# Autodesk Inventor assembly: ude
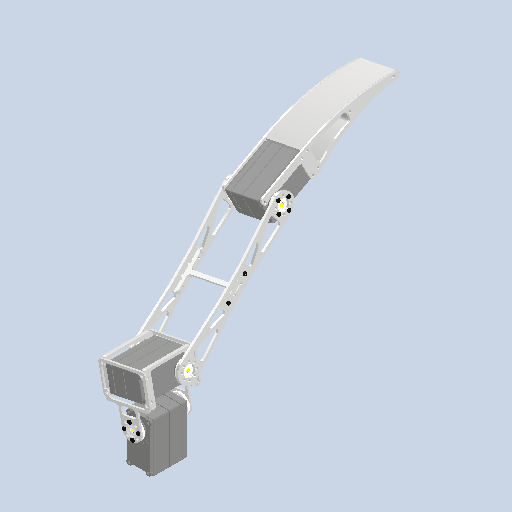
[picture p0: Inventor's stored thumbnail of the model, 512x512]
Saved by Autodesk Inventor 2024 (Build 280153000, 153)
## iProperties
Created: 2023-03-29
Part Number: ude
Document SubType Name: Assembly
Designer: right
Mass: 174.923 g
Surface Area: 565.861 cm^2
Volume: 110.018 cm^3
Density: 1.58994 g/cm^3
Author: right
## Documents named in this file (11)
- C:\Users\right\OneDrive\ドキュメント\Inventor\V2二足Light＿仮\ude.iam
- C:\Users\right\OneDrive\ドキュメント\Inventor\V2二足Light＿仮\KRS2500_scale.ipt
- C:\Users\right\OneDrive\ドキュメント\Inventor\V2二足Light＿仮\02157_SmallDiameterHornB.ipt
- C:\Users\right\OneDrive\ドキュメント\Inventor\V2二足Light＿仮\kata.ipt
- C:\Users\right\OneDrive\ドキュメント\Inventor\V2二足Light＿仮\腕.ipt
- C:\Users\right\OneDrive\ドキュメント\Inventor\V2二足Light＿仮\腕の筋交い.ipt
- C:\Users\right\OneDrive\ドキュメント\Inventor\V2二足Light＿仮\02159_SmallFreeHornC.ipt
- C:\Users\right\OneDrive\ドキュメント\Inventor\V2二足Light＿仮\hand.ipt
- C:\Users\right\OneDrive\ドキュメント\Inventor\V2二足Light＿仮\M2小ねじ.ipt
- C:\Users\right\OneDrive\ドキュメント\Inventor\V2二足Light＿仮\上腕.ipt
- C:\Users\right\OneDrive\ドキュメント\Inventor\V2二足Light＿仮\sphand2.ipt
## Components (35 placed, 10 different names)
1. KRS2500_scale:1 — 挿入:1, 挿入:63
2. 02157_SmallDiameterHornB:1 — 挿入:1, 挿入:4, 挿入:5
3. kata:1 — 挿入:4, 挿入:5, 挿入:53, 挿入:54, 挿入:55, 挿入:56, 挿入:66, 挿入:67, 挿入:71
4. KRS2500_scale:2 — 挿入:17, 挿入:69, 挿入:70, 挿入:73, 挿入:74
5. 02157_SmallDiameterHornB:2 — 挿入:15, 挿入:16
6. 腕:1 — 挿入:18, 挿入:19, 挿入:20, 挿入:21, 挿入:27, 挿入:28, 挿入:43, 挿入:44, 挿入:49, 挿入:50, 挿入:51, 挿入:52
7. 腕:2 — 挿入:15, 挿入:16, 挿入:22, 挿入:25, 挿入:26, 挿入:37, 挿入:38, 挿入:39, 挿入:40, 挿入:41, 挿入:42
8. 腕の筋交い:1 — 挿入:20, 挿入:21, 挿入:22
9. 02159_SmallFreeHornC:1 — 挿入:17, 挿入:18, 挿入:19
10. KRS2500_scale:3 — 挿入:29, 挿入:30, 挿入:31, 挿入:32
11. 02157_SmallDiameterHornB:3 — 挿入:25, 挿入:26
12. 02159_SmallFreeHornC:2 — 挿入:27, 挿入:28
13. hand:1 — 挿入:29, 挿入:30, フラッシュ:1, 挿入:75
14. hand:2 — 挿入:31, 挿入:32, 挿入:76
15. M2小ねじ:2 — 挿入:52
16. M2小ねじ:3 — 挿入:37
17. M2小ねじ:4 — 挿入:38
18. M2小ねじ:7 — 挿入:49
19. M2小ねじ:8 — 挿入:50
20. M2小ねじ:10 — 挿入:44
21. M2小ねじ:12 — 挿入:51
22. M2小ねじ:13 — 挿入:40
23. M2小ねじ:14 — 挿入:41
24. M2小ねじ:18 — 挿入:42
25. M2小ねじ:19 — 挿入:43
26. M2小ねじ:20 — 挿入:39
27. M2小ねじ:21 — 挿入:56
28. M2小ねじ:22 — 挿入:55
29. M2小ねじ:23 — 挿入:54
30. M2小ねじ:24 — 挿入:53
31. 02159_SmallFreeHornC:3 — 挿入:63, 挿入:64, 挿入:65
32. kata:2 — 挿入:64, 挿入:65, 挿入:68, 挿入:72
33. 上腕:1 — 挿入:66, 挿入:67, 挿入:68, 挿入:69, 挿入:70
34. 上腕:2 — 挿入:71, 挿入:72, 挿入:73, 挿入:74
35. sphand2:1 — フラッシュ:1, 挿入:75, 挿入:76
## Relationships (53: Insert 52, Flush 1)
- 挿入:1 [Insert]: KRS2500_scale:1 ↔ 02157_SmallDiameterHornB:1
- 挿入:4 [Insert]: 02157_SmallDiameterHornB:1 ↔ kata:1
- 挿入:5 [Insert]: 02157_SmallDiameterHornB:1 ↔ kata:1
- [Insert]: KRS2500_scale:2 ↔ 02157_SmallDiameterHornB:2
- 挿入:15 [Insert]: 02157_SmallDiameterHornB:2 ↔ 腕:2
- 挿入:16 [Insert]: 02157_SmallDiameterHornB:2 ↔ 腕:2
- 挿入:17 [Insert]: KRS2500_scale:2 ↔ 02159_SmallFreeHornC:1
- 挿入:18 [Insert]: 腕:1 ↔ 02159_SmallFreeHornC:1
- 挿入:19 [Insert]: 腕:1 ↔ 02159_SmallFreeHornC:1
- 挿入:20 [Insert]: 腕:1 ↔ 腕の筋交い:1
- 挿入:21 [Insert]: 腕:1 ↔ 腕の筋交い:1
- 挿入:22 [Insert]: 腕:2 ↔ 腕の筋交い:1
- [Insert]: KRS2500_scale:3 ↔ 02157_SmallDiameterHornB:3
- [Insert]: KRS2500_scale:3 ↔ 02159_SmallFreeHornC:2
- 挿入:25 [Insert]: 腕:2 ↔ 02157_SmallDiameterHornB:3
- 挿入:26 [Insert]: 腕:2 ↔ 02157_SmallDiameterHornB:3
- 挿入:27 [Insert]: 腕:1 ↔ 02159_SmallFreeHornC:2
- 挿入:28 [Insert]: 腕:1 ↔ 02159_SmallFreeHornC:2
- 挿入:29 [Insert]: KRS2500_scale:3 ↔ hand:1
- 挿入:30 [Insert]: KRS2500_scale:3 ↔ hand:1
- 挿入:31 [Insert]: KRS2500_scale:3 ↔ hand:2
- 挿入:32 [Insert]: KRS2500_scale:3 ↔ hand:2
- 挿入:37 [Insert]: 腕:2 ↔ M2小ねじ:3
- 挿入:38 [Insert]: 腕:2 ↔ M2小ねじ:4
- 挿入:39 [Insert]: 腕:2 ↔ M2小ねじ:20
- 挿入:40 [Insert]: 腕:2 ↔ M2小ねじ:13
- 挿入:41 [Insert]: 腕:2 ↔ M2小ねじ:14
- 挿入:42 [Insert]: 腕:2 ↔ M2小ねじ:18
- 挿入:43 [Insert]: 腕:1 ↔ M2小ねじ:19
- 挿入:44 [Insert]: 腕:1 ↔ M2小ねじ:10
- 挿入:49 [Insert]: 腕:1 ↔ M2小ねじ:7
- 挿入:50 [Insert]: 腕:1 ↔ M2小ねじ:8
- 挿入:51 [Insert]: 腕:1 ↔ M2小ねじ:12
- 挿入:52 [Insert]: 腕:1 ↔ M2小ねじ:2
- 挿入:53 [Insert]: kata:1 ↔ M2小ねじ:24
- 挿入:54 [Insert]: kata:1 ↔ M2小ねじ:23
- 挿入:55 [Insert]: kata:1 ↔ M2小ねじ:22
- 挿入:56 [Insert]: kata:1 ↔ M2小ねじ:21
- 挿入:63 [Insert]: KRS2500_scale:1 ↔ 02159_SmallFreeHornC:3
- 挿入:64 [Insert]: 02159_SmallFreeHornC:3 ↔ kata:2
- 挿入:65 [Insert]: 02159_SmallFreeHornC:3 ↔ kata:2
- 挿入:66 [Insert]: kata:1 ↔ 上腕:1
- 挿入:67 [Insert]: kata:1 ↔ 上腕:1
- 挿入:68 [Insert]: kata:2 ↔ 上腕:1
- 挿入:69 [Insert]: KRS2500_scale:2 ↔ 上腕:1
- 挿入:70 [Insert]: KRS2500_scale:2 ↔ 上腕:1
- 挿入:71 [Insert]: kata:1 ↔ 上腕:2
- 挿入:72 [Insert]: kata:2 ↔ 上腕:2
- 挿入:73 [Insert]: KRS2500_scale:2 ↔ 上腕:2
- 挿入:74 [Insert]: KRS2500_scale:2 ↔ 上腕:2
- フラッシュ:1 [Flush]: hand:1 ↔ sphand2:1
- 挿入:75 [Insert]: hand:1 ↔ sphand2:1
- 挿入:76 [Insert]: hand:2 ↔ sphand2:1
## Named parameters: d9_d0 = 0 mm, d22_d9_d0 = 0 mm, d23_d16 = 0 mm
